# Autodesk Inventor assembly: 66_100_rail+mount
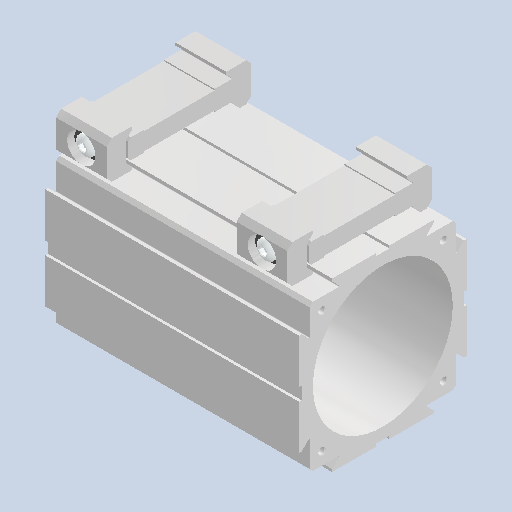
[picture p0: Inventor's stored thumbnail of the model, 512x512]
Saved by Autodesk Inventor 2026.1 (Build 301233000, 233)
## iProperties
Created: 2019-04-24
Part Number: 66_100_rail+mount
Document SubType Name: Assembly
Designer: Administrator
Author: Administrator
## Documents named in this file (3)
- C:\Users\user\Desktop\setup_inventor_2025\LightPath\66_100_rail+mount.iam
- C:\Users\user\Desktop\setup_inventor_2025\LightPath\XT66-66mm-rail-100.ipt
- C:\Users\user\Desktop\setup_inventor_2025\LightPath\XT66C1-66mm_railmount_short.ipt
## Components (3 placed, 2 different names)
1. XT66-66mm-rail-100:1 — Mate:1, Flush:1, Mate:2, Flush:2, Flush:3, Flush:4
2. XT66C1-66mm_railmount_short:1 — Mate:1, Flush:1, Flush:4
3. XT66C1-66mm_railmount_short:2 — Mate:2, Flush:2, Flush:3
## Relationships (6: Flush 4, Mate 2)
- Mate:1: XT66-66mm-rail-100:1 ↔ XT66C1-66mm_railmount_short:1
- Flush:1: XT66-66mm-rail-100:1 ↔ XT66C1-66mm_railmount_short:1
- Mate:2: XT66-66mm-rail-100:1 ↔ XT66C1-66mm_railmount_short:2
- Flush:2: XT66-66mm-rail-100:1 ↔ XT66C1-66mm_railmount_short:2
- Flush:3: XT66-66mm-rail-100:1 ↔ XT66C1-66mm_railmount_short:2
- Flush:4 (8.81 mm): XT66-66mm-rail-100:1 ↔ XT66C1-66mm_railmount_short:1
